# Autodesk Inventor assembly: one side of drive
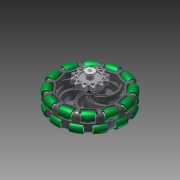
[picture p0: Inventor's stored thumbnail of the model, 180x180]
Saved by Autodesk Inventor 2014 SP1 (Build 180222100, 222)
## iProperties
Created: 2013-10-05
Part Number: one side of drive
Document SubType Name: Assembly
Designer: RyanHughes
Author: RyanHughes
## Documents named in this file (6)
- C:\Users\Ryan\Desktop\sw\toss up 2ed A bot\drivetrain\wheel asmby.iam
- C:\Users\Ryan\Desktop\sw\lib\Super Sonic Sparks VEX CAD Library\Wheels\4'' Omni-Directional Wheel.iam
- C:\Users\Ryan\Desktop\sw\lib\Aperture VEX CAD Library\Shaft\2 inch Shaft.ipt
- C:\Users\Ryan\Desktop\sw\lib\Aperture VEX CAD Library\Sprockets\HS Sprockets\12 Tooth HS Sprocket.ipt
- C:\Users\Ryan\Desktop\sw\lib\Aperture VEX CAD Library\Spacers\SPACER-0500-0125.ipt
- C:\Users\Ryan\Desktop\sw\lib\Aperture VEX CAD Library\Hardware\Shaft Collar.ipt
## Components (5 placed, 5 different names)
1. 2 inch Shaft:1 — Mate:216, Mate:217, Flush:1
2. 12 Tooth HS Sprocket:1 — Mate:210, Mate:211, Mate:212, Mate:213, Mate:215, Mate:216, Mate:217
3. 4'' Omni-Directional Wheel:1 [sub-assembly] — Mate:214, Mate:215, Flush:1
4. SPACER-0500-0125:3 — Mate:210, Mate:211
5. Shaft Collar:1 — Mate:212, Mate:213, Mate:214
## Relationships (9: Mate 8, Flush 1)
- Mate:210: 12 Tooth HS Sprocket:1 ↔ SPACER-0500-0125:3
- Mate:211: 12 Tooth HS Sprocket:1 ↔ SPACER-0500-0125:3
- Mate:212: 12 Tooth HS Sprocket:1 ↔ Shaft Collar:1
- Mate:213: 12 Tooth HS Sprocket:1 ↔ Shaft Collar:1
- Mate:214: 4'' Omni-Directional Wheel:1 ↔ Shaft Collar:1
- Mate:215: 12 Tooth HS Sprocket:1 ↔ 4'' Omni-Directional Wheel:1
- Mate:216: 2 inch Shaft:1 ↔ 12 Tooth HS Sprocket:1
- Mate:217: 2 inch Shaft:1 ↔ 12 Tooth HS Sprocket:1
- Flush:1 (-6.35 mm): 2 inch Shaft:1 ↔ 4'' Omni-Directional Wheel:1
